# Autodesk Inventor assembly: Lamiere e sensore ultrasuoni - Trasporto
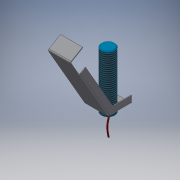
[picture p0: Inventor's stored thumbnail of the model, 180x180]
Saved by Autodesk Inventor 2018 (Build 220112000, 112)
## iProperties
Created: 2020-06-12
Part Number: Lamiere e sensore ultrasuoni - Trasporto
Material: Generico
Document SubType Name: Assembly
Designer: Francesco
Author: Francesco
## Documents named in this file (3)
- C:\Users\Francesco\no-brim\Meccanica\Progetto Inventor no-brim\Assiemi\Lamiere e sensore ultrasuoni - Trasporto.iam
- C:\Users\Francesco\no-brim\Meccanica\Progetto Inventor no-brim\Parti\Modello sensore ultrasuoni.ipt
- C:\Users\Francesco\no-brim\Meccanica\Progetto Inventor no-brim\Parti\Lamiera supporto ultrasuoni.ipt
## Components (2 placed, 2 different names)
1. Modello sensore ultrasuoni:1 — Coincidente:1, Allineato:1
2. Lamiera supporto ultrasuoni:1 — Coincidente:1, Allineato:1
## Relationships (2: Mate 1, Flush 1)
- Coincidente:1 [Mate]: Modello sensore ultrasuoni:1 ↔ Lamiera supporto ultrasuoni:1
- Allineato:1 [Flush] (-10 mm): Modello sensore ultrasuoni:1 ↔ Lamiera supporto ultrasuoni:1
